# Autodesk Inventor assembly: Case
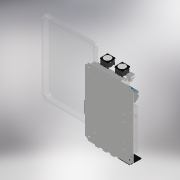
[picture p0: Inventor's stored thumbnail of the model, 180x180]
Saved by Autodesk Inventor 2020 (Build 240168000, 168)
## iProperties
Created: 2019-12-11
Part Number: Case
Document SubType Name: Assembly
Designer: nicoc
Author: nicoc
## Documents named in this file (14)
- D:\repos\_finished\P5-AIonFPGA\cad\Case\Case.iam
- D:\repos\_finished\P5-AIonFPGA\cad\Case\Ultra96\PWB_USDEV1-1_FINAL.iam
- D:\repos\_finished\P5-AIonFPGA\cad\Case\Terminalblock\Terminalblock.iam
- D:\repos\_finished\P5-AIonFPGA\cad\Case\SlottedWiring\SlottexWiring200mm.ipt
- D:\repos\_finished\P5-AIonFPGA\cad\Case\SlottedWiring\SlottexWiring110mm.ipt
- D:\repos\_finished\P5-AIonFPGA\cad\Case\Fibox_PC_3828 _3_T_Bottom.ipt
- D:\repos\_finished\P5-AIonFPGA\cad\Case\Fibox_PC_3828 _3_T_Top.ipt
- D:\repos\_finished\P5-AIonFPGA\cad\Case\Ventilator\Fan_40x40x20.iam
- D:\repos\_finished\P5-AIonFPGA\cad\Case\Ventilator\Fan_60x60x25.ipt
- D:\repos\_finished\P5-AIonFPGA\cad\Case\Ultra96\USBCable.ipt
- D:\repos\_finished\P5-AIonFPGA\cad\Case\Ventilator\Filter40x40.ipt
- D:\repos\_finished\P5-AIonFPGA\cad\Case\QuickCableGlandes\QuickCableGlandes.ipt
- D:\repos\_finished\P5-AIonFPGA\cad\Case\Ventilator\Filter60x60.ipt
- D:\repos\_finished\P5-AIonFPGA\cad\Case\MetalSheet.ipt
## Components (20 placed, 13 different names)
1. PWB_USDEV1-1_FINAL:1 [sub-assembly] — Mate:23, Flush:20, Flush:21, Mate:36, Flush:35, Flush:39
2. Terminalblock:1 [sub-assembly] — Mate:37, Flush:37, Flush:38
3. SlottexWiring200mm:1 — Mate:33, Flush:29, Flush:30, Mate:34, Flush:31, Flush:32
4. SlottexWiring200mm:2 — Mate:35, Flush:33, Flush:34
5. SlottexWiring110mm:1 — Mate:34, Flush:31, Flush:32, Mate:35, Flush:33, Flush:34
6. Fibox_PC_3828 _3_T_Bottom:1 — Mate:21, Mate:27, Mate:28, Mate:29, Mate:30, Tangent:3, Tangent:4, Tangent:5, Mate:31, Mate:32, Mate:38, Mate:39, Mate:40, Mate:41
7. Fibox_PC_3828 _3_T_Top:1 — Mate:21
8. Fan_40x40x20:1 [sub-assembly]
9. Fan_40x40x20:3 [sub-assembly]
10. Fan_60x60x25:1 — Flush:27, Flush:28
11. USBCable:1 — Mate:23, Flush:20, Flush:21
12. Filter40x40:1
13. Filter40x40:2
14. QuickCableGlandes:1 — Mate:27
15. QuickCableGlandes:2 — Mate:28, Tangent:4
16. QuickCableGlandes:3 — Mate:29, Tangent:5
17. QuickCableGlandes:4 — Mate:30, Tangent:3
18. Filter60x60:1 — Mate:32
19. Filter60x60:2 — Mate:31, Flush:27, Flush:28
20. MetalSheet:1 — Mate:33, Flush:29, Flush:30, Mate:36, Flush:35, Mate:37, Flush:37, Flush:38, Mate:38, Mate:39, Mate:40, Mate:41, Flush:39
## Relationships (34: Mate 17, Flush 14, Tangent 3)
- Mate:21: Fibox_PC_3828 _3_T_Bottom:1 ↔ Fibox_PC_3828 _3_T_Top:1
- Mate:23: PWB_USDEV1-1_FINAL:1 ↔ USBCable:1
- Flush:20: PWB_USDEV1-1_FINAL:1 ↔ USBCable:1
- Flush:21 (1 mm): PWB_USDEV1-1_FINAL:1 ↔ USBCable:1
- Mate:27: Fibox_PC_3828 _3_T_Bottom:1 ↔ QuickCableGlandes:1
- Mate:28: Fibox_PC_3828 _3_T_Bottom:1 ↔ QuickCableGlandes:2
- Mate:29: Fibox_PC_3828 _3_T_Bottom:1 ↔ QuickCableGlandes:3
- Mate:30: Fibox_PC_3828 _3_T_Bottom:1 ↔ QuickCableGlandes:4
- Tangent:3: Fibox_PC_3828 _3_T_Bottom:1 ↔ QuickCableGlandes:4
- Tangent:4: Fibox_PC_3828 _3_T_Bottom:1 ↔ QuickCableGlandes:2
- Tangent:5: Fibox_PC_3828 _3_T_Bottom:1 ↔ QuickCableGlandes:3
- Mate:31: Fibox_PC_3828 _3_T_Bottom:1 ↔ Filter60x60:2
- Mate:32: Fibox_PC_3828 _3_T_Bottom:1 ↔ Filter60x60:1
- Flush:27: Fan_60x60x25:1 ↔ Filter60x60:2
- Flush:28: Fan_60x60x25:1 ↔ Filter60x60:2
- Mate:33: SlottexWiring200mm:1 ↔ MetalSheet:1
- Flush:29 (25 mm): SlottexWiring200mm:1 ↔ MetalSheet:1
- Flush:30 (114 mm): SlottexWiring200mm:1 ↔ MetalSheet:1
- Mate:34: SlottexWiring200mm:1 ↔ SlottexWiring110mm:1
- Flush:31: SlottexWiring200mm:1 ↔ SlottexWiring110mm:1
- Flush:32: SlottexWiring200mm:1 ↔ SlottexWiring110mm:1
- Mate:35: SlottexWiring200mm:2 ↔ SlottexWiring110mm:1
- Flush:33: SlottexWiring200mm:2 ↔ SlottexWiring110mm:1
- Flush:34: SlottexWiring200mm:2 ↔ SlottexWiring110mm:1
- Mate:36: PWB_USDEV1-1_FINAL:1 ↔ MetalSheet:1
- Flush:35 (97.5 mm): PWB_USDEV1-1_FINAL:1 ↔ MetalSheet:1
- Mate:37: Terminalblock:1 ↔ MetalSheet:1
- Flush:37 (13.5 mm): Terminalblock:1 ↔ MetalSheet:1
- Flush:38 (40.5 mm): Terminalblock:1 ↔ MetalSheet:1
- Mate:38: Fibox_PC_3828 _3_T_Bottom:1 ↔ MetalSheet:1
- Mate:39: Fibox_PC_3828 _3_T_Bottom:1 ↔ MetalSheet:1
- Mate:40 (-13.25 mm): Fibox_PC_3828 _3_T_Bottom:1 ↔ MetalSheet:1
- Mate:41 (-13.25 mm): Fibox_PC_3828 _3_T_Bottom:1 ↔ MetalSheet:1
- Flush:39 (175 mm): PWB_USDEV1-1_FINAL:1 ↔ MetalSheet:1
